# Autodesk Inventor assembly: rocket_asm_2
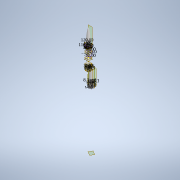
[picture p0: Inventor's stored thumbnail of the model, 180x180]
Saved by Autodesk Inventor 2020 (Build 240168000, 168)
## iProperties
Created: 2022-05-22
Part Number: rocket_asm_2
Document SubType Name: Assembly
Designer: sp
Author: sp
## Documents named in this file (8)
- C:\Users\sp\Documents\Rocket\rocket\CAD\rocket_asm_2.iam
- C:\Users\sp\Documents\Rocket\rocket\CAD\Spitze.ipt
- C:\Users\sp\Documents\Rocket\rocket\CAD\Cam_konstruction.ipt
- C:\Users\sp\Documents\Rocket\rocket\CAD\Segment_elektro.ipt
- C:\Users\sp\Documents\Rocket\rocket\CAD\Elektro_asm.iam
- C:\Users\sp\Documents\Rocket\rocket\CAD\Servo_Ku_asm.iam
- C:\Users\sp\Documents\Rocket\rocket\CAD\Segment_mitte.ipt
- C:\Users\sp\Documents\Rocket\rocket\CAD\recovery_structure2_asm.iam
## Components (7 placed, 7 different names)
1. Spitze:1 — Einfügen:1, Passend:1
2. Cam_konstruction:1 — Einfügen:1, Passend:1, Einfügen:2, Passend:2
3. Segment_elektro:1 — Einfügen:2, Passend:2, Einfügen:4
4. Elektro_asm:1 [sub-assembly] — Einfügen:3, Passend:3
5. Servo_Ku_asm:1 [sub-assembly] — Einfügen:3, Passend:3, Einfügen:4
6. Segment_mitte:1 — Einfügen:5
7. recovery_structure2_asm:1 [sub-assembly] — Einfügen:5
## Relationships (8: Insert 5, Mate 3)
- Einfügen:1 [Insert]: Spitze:1 ↔ Cam_konstruction:1
- Passend:1 [Mate]: Spitze:1 ↔ Cam_konstruction:1
- Einfügen:2 [Insert]: Cam_konstruction:1 ↔ Segment_elektro:1
- Passend:2 [Mate]: Cam_konstruction:1 ↔ Segment_elektro:1
- Einfügen:3 [Insert] (10 mm): Elektro_asm:1 ↔ Servo_Ku_asm:1
- Passend:3 [Mate]: Elektro_asm:1 ↔ Servo_Ku_asm:1
- Einfügen:4 [Insert]: Segment_elektro:1 ↔ Servo_Ku_asm:1
- Einfügen:5 [Insert]: Segment_mitte:1 ↔ recovery_structure2_asm:1
